# Autodesk Inventor assembly: motor_MIROR
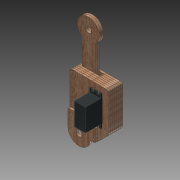
[picture p0: Inventor's stored thumbnail of the model, 180x180]
Saved by Autodesk Inventor 2015 (Build 190159000, 159)
## iProperties
Created: 2016-02-03
Part Number: motor_MIROR
Document SubType Name: Assembly
Designer: david
Author: david
## Documents named in this file (10)
- Z:\gip\Inventor\generatie 7\motor v2\motor_MIROR.iam
- Z:\gip\Inventor\generatie 7\motor v2\p1_MIROR.ipt
- Z:\gip\Inventor\generatie 7\motor v2\p2_MIROR.ipt
- Z:\gip\Inventor\generatie 7\motor v2\p3_MIROR.ipt
- Z:\gip\Inventor\generatie 7\motor v2\p5_MIROR.ipt
- Z:\gip\Inventor\generatie 7\motor v2\servo\block_MIROR.ipt
- Z:\gip\Inventor\generatie 7\motor v2\servo\tang_MIROR.ipt
- Z:\gip\Inventor\generatie 7\old\Motor\tanden2_MIROR.ipt
- Z:\gip\Inventor\generatie 7\motor v2\tandwiel\tandwiel_MIROR.iam
- Z:\gip\Inventor\generatie 7\motor v2\p6_MIROR.ipt
## Components (13 placed, 9 different names)
1. p1_MIROR:1 — Flush:2, Mate:1, Flush:16, Flush:4, Flush:18
2. p2_MIROR:1 — Flush:2, Mate:1, Mate:22, Mate:2, Flush:5
3. p2_MIROR:2 — Flush:16, Mate:22, Flush:4, Mate:2, Mate:23, Mate:3, Mate:15, Mate:21, Flush:20
4. p3_MIROR:1 — Mate:23, Flush:5, Mate:3, Mate:13, Mate:33, Mate:32
5. p5_MIROR:1 — Flush:18, Mate:31, Mate:30, Mate:29, Mate:37, Flush:22, Mate:36, Mate:40, Mate:39, Mate:38
6. block_MIROR:1 — Mate:31, Mate:30, Mate:29, Mate:11, Mate:10
7. tang_MIROR:1 — Mate:11, Mate:10, Mate:18, Mate:16
8. tanden2_MIROR:1 — Mate:15, Mate:13, Rotation/Translation:1, Mate:20, Flush:13, Mate:19
9. tandwiel_MIROR:1 [sub-assembly] — Mate:18, Mate:16, Rotation/Translation:1, Flush:19
10. tanden2_MIROR:2 — Flush:19, Mate:21, Mate:20, Flush:13, Mate:19
11. p3_MIROR:2 — Mate:33, Flush:20, Mate:32, Mate:35, Flush:21, Mate:34
12. p3_MIROR:3 — Mate:37, Flush:22, Mate:36, Mate:35, Flush:21, Mate:34
13. p6_MIROR:1 — Mate:40, Mate:39, Mate:38
## Relationships (37: Mate 26, Flush 10, RelateRotateTranslate 1)
- Flush:2: p1_MIROR:1 ↔ p2_MIROR:1
- Mate:1: p1_MIROR:1 ↔ p2_MIROR:1
- Flush:16: p1_MIROR:1 ↔ p2_MIROR:2
- Mate:22: p2_MIROR:1 ↔ p2_MIROR:2
- Flush:4: p1_MIROR:1 ↔ p2_MIROR:2
- Mate:2: p2_MIROR:1 ↔ p2_MIROR:2
- Mate:23: p2_MIROR:2 ↔ p3_MIROR:1
- Flush:5: p2_MIROR:1 ↔ p3_MIROR:1
- Mate:3: p2_MIROR:2 ↔ p3_MIROR:1
- Flush:18: p1_MIROR:1 ↔ p5_MIROR:1
- Mate:31: p5_MIROR:1 ↔ block_MIROR:1
- Mate:30: p5_MIROR:1 ↔ block_MIROR:1
- Mate:29: p5_MIROR:1 ↔ block_MIROR:1
- Mate:11: block_MIROR:1 ↔ tang_MIROR:1
- Mate:10: block_MIROR:1 ↔ tang_MIROR:1
- Mate:15: p2_MIROR:2 ↔ tanden2_MIROR:1
- Mate:13: p3_MIROR:1 ↔ tanden2_MIROR:1
- Mate:18: tang_MIROR:1 ↔ tandwiel_MIROR:1
- Mate:16 (0.15 mm): tang_MIROR:1 ↔ tandwiel_MIROR:1
- Rotation/Translation:1 [RelateRotateTranslate] (100 mm): tanden2_MIROR:1 ↔ tandwiel_MIROR:1
- Flush:19: tandwiel_MIROR:1 ↔ tanden2_MIROR:2
- Mate:21: p2_MIROR:2 ↔ tanden2_MIROR:2
- Mate:20: tanden2_MIROR:1 ↔ tanden2_MIROR:2
- Flush:13: tanden2_MIROR:1 ↔ tanden2_MIROR:2
- Mate:19: tanden2_MIROR:1 ↔ tanden2_MIROR:2
- Mate:33: p3_MIROR:1 ↔ p3_MIROR:2
- Flush:20: p2_MIROR:2 ↔ p3_MIROR:2
- Mate:32: p3_MIROR:1 ↔ p3_MIROR:2
- Mate:37: p5_MIROR:1 ↔ p3_MIROR:3
- Flush:22: p5_MIROR:1 ↔ p3_MIROR:3
- Mate:36: p5_MIROR:1 ↔ p3_MIROR:3
- Mate:35: p3_MIROR:2 ↔ p3_MIROR:3
- Flush:21: p3_MIROR:2 ↔ p3_MIROR:3
- Mate:34: p3_MIROR:2 ↔ p3_MIROR:3
- Mate:40: p5_MIROR:1 ↔ p6_MIROR:1
- Mate:39: p5_MIROR:1 ↔ p6_MIROR:1
- Mate:38: p5_MIROR:1 ↔ p6_MIROR:1
